# Autodesk Inventor assembly: Ensamblaje del tambor con sis. Lebus
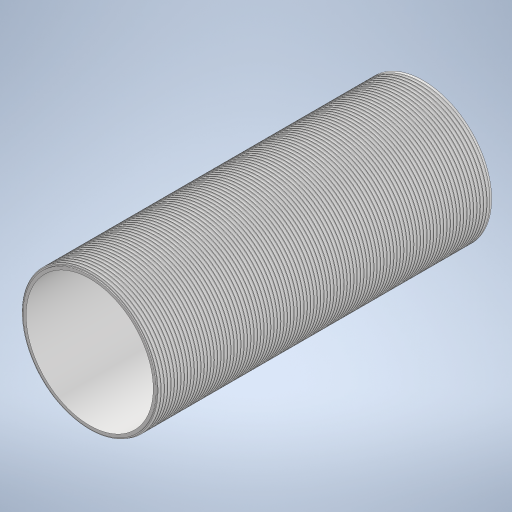
[picture p0: Inventor's stored thumbnail of the model, 512x512]
Saved by Autodesk Inventor 2024.3 (Build 283343000, 343)
## iProperties
Created: 2025-07-06
Part Number: Ensamblaje del tambor con sis. Lebus
Document SubType Name: Assembly
Designer: Daniel Rodriguez
Author: Daniel Rodriguez
## Documents named in this file (3)
- C:\Users\Daniel Rodriguez\Downloads\winch-drum-welding-assembly\Nuestro Winch\Ensamblaje del tambor con sis. Lebus.iam
- C:\Users\Daniel Rodriguez\Downloads\winch-drum-welding-assembly\Nuestro Winch\Tambor liso (drum).ipt
- C:\Users\Daniel Rodriguez\Downloads\winch-drum-welding-assembly\Nuestro Winch\Sistema LEBUS.ipt
## Components (2 placed, 2 different names)
1. Tambor liso (drum):1 — Coincidencia:1, Coincidencia:2, Coincidencia:3
2. Sistema LEBUS:1 — Coincidencia:2, Coincidencia:3
## Relationships (3: Mate 3)
- Coincidencia:1 [Mate]: Tambor liso (drum):1
- Coincidencia:2 [Mate]: Tambor liso (drum):1 ↔ Sistema LEBUS:1
- Coincidencia:3 [Mate]: Tambor liso (drum):1 ↔ Sistema LEBUS:1
